# Autodesk Inventor assembly: roots_blower_1
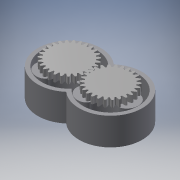
[picture p0: Inventor's stored thumbnail of the model, 180x180]
Saved by Autodesk Inventor 2018.3 (Build 223284000, 284)
## iProperties
Created: 2021-03-20
Part Number: roots_blower_1
Document SubType Name: Assembly
Designer: kenbl
Author: kenbl
## Documents named in this file (4)
- C:\Users\kenbl\OneDrive\Documents\School\sd\roots\roots_blower_1.iam
- C:\Users\kenbl\OneDrive\Documents\School\sd\roots_rotor_3lobe.ipt
- C:\Users\kenbl\OneDrive\Documents\School\sd\housing.ipt
- C:\Users\kenbl\OneDrive\Documents\School\sd\roots\roots_blower_1\Design Accelerator\Spur Gears2.iam
## Components (4 placed, 3 different names)
1. roots_rotor_3lobe:1 — Rotational:2, Mate:2
2. roots_rotor_3lobe:2 — Rotational:1
3. housing:1 — Rotational:1, Rotational:2, Mate:1, Mate:3
4. Spur Gears:1 [sub-assembly] — Mate:1, Mate:2, Mate:3
## Relationships (5: Mate 3, RevoluteJoint 2)
- Rotational:1 [RevoluteJoint]: roots_rotor_3lobe:2 ↔ housing:1
- Rotational:2 [RevoluteJoint]: roots_rotor_3lobe:1 ↔ housing:1
- Mate:1: housing:1 ↔ Spur Gears:1
- Mate:2: roots_rotor_3lobe:1 ↔ Spur Gears:1
- Mate:3: housing:1 ↔ Spur Gears:1
